# Autodesk Inventor assembly: finger-assembly
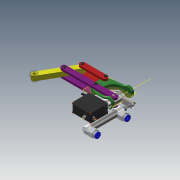
[picture p0: Inventor's stored thumbnail of the model, 180x180]
Saved by Autodesk Inventor 2017 (Build 210142000, 142)
## iProperties
Created: 2018-05-30
Part Number: finger-assembly
Document SubType Name: Assembly
Designer: Luiz Gustavo
Author: Luiz Gustavo
## Documents named in this file (14)
- C:\Users\Luiz Gustavo\Documents\Inventor\piano-robot\finger-assembly.iam
- C:\Users\Luiz Gustavo\Documents\Inventor\piano-robot\fingers-reference.ipt
- C:\Users\Luiz Gustavo\Documents\Inventor\piano-robot\biela-dedo-1.ipt
- C:\Users\Luiz Gustavo\Documents\Inventor\piano-robot\biela-dedo-2.ipt
- C:\Users\Luiz Gustavo\Documents\Inventor\piano-robot\biela-dedo-3.ipt
- C:\Users\Luiz Gustavo\Documents\Inventor\piano-robot\bloco-dedo-1.ipt
- C:\Users\Luiz Gustavo\Documents\Inventor\piano-robot\slider-1.ipt
- C:\Users\Luiz Gustavo\Documents\Inventor\piano-robot\tgy-901d.ipt
- C:\Users\Luiz Gustavo\Documents\Inventor\piano-robot\garfo-1.ipt
- C:\Users\Luiz Gustavo\Documents\Inventor\piano-robot\cylinderAssembly.iam
- C:\Users\Luiz Gustavo\Documents\Inventor\piano-robot\tip-protector.ipt
- C:\Users\Luiz Gustavo\Documents\Inventor\piano-robot\grabcad\AIRTAC 4V21008\PC602.ipt
- C:\Users\Luiz Gustavo\Documents\Inventor\piano-robot\finger-assembly\Design Accelerator\Bolted Connection1.iam
- C:\Users\Luiz Gustavo\Documents\Inventor\piano-robot\servo-metal-arm.ipt
## Components (14 placed, 13 different names)
1. fingers-reference:1 — Mate:1
2. biela-dedo-1:1 — Flush:1, Rotational:4, Rotational:5, Rigid:7
3. biela-dedo-2:1 — Flush:2, Rotational:3, Rotational:4, Mate:12, Mate:13
4. biela-dedo-3:1 — Flush:3, Rotational:2, Rotational:5, Transitional:1
5. bloco-dedo-1:1 — Flush:4, Rotational:2, Rotational:3, Mate:3, Mate:9, Mate:10
6. slider-1:1 — Mate:2, Flush:5, Mate:3, Rotational:6, Transitional:1
7. tgy-901d:1 — Mate:4, Angle:1, Flush:6, Mate:5
8. garfo-1:1 — Rigid:6, Rotational:6
9. cylinderAssembly:1 [sub-assembly] — Mate:5, Flush:7, Rigid:6, Rigid:8, Rigid:9
10. tip-protector:1 — Rigid:7
11. PC602:1 — Rigid:8
12. PC602:2 — Rigid:9
13. Bolted Connection:1 [sub-assembly] — Mate:12, Mate:13
14. servo-metal-arm:1 — Mate:9, Mate:10, Mate:11
## Relationships (28: Mate 10, Flush 7, RevoluteJoint 5, WeldJoint 4, Angle 1, Transitional 1)
- Flush:1: biela-dedo-1:1
- Flush:2: biela-dedo-2:1
- Flush:3: biela-dedo-3:1
- Flush:4: bloco-dedo-1:1
- Rotational:2 [RevoluteJoint]: biela-dedo-3:1 ↔ bloco-dedo-1:1
- Rotational:3 [RevoluteJoint]: biela-dedo-2:1 ↔ bloco-dedo-1:1
- Rotational:4 [RevoluteJoint]: biela-dedo-1:1 ↔ biela-dedo-2:1
- Rotational:5 [RevoluteJoint]: biela-dedo-1:1 ↔ biela-dedo-3:1
- Mate:1: fingers-reference:1
- Mate:2: slider-1:1
- Flush:5: slider-1:1
- Mate:3: bloco-dedo-1:1 ↔ slider-1:1
- Mate:4: tgy-901d:1
- Angle:1 (180 deg): tgy-901d:1
- Flush:6 (39.1 mm): tgy-901d:1
- Mate:5: tgy-901d:1 ↔ cylinderAssembly:1
- Flush:7 (48 mm): cylinderAssembly:1
- Rigid:6 [WeldJoint]: garfo-1:1 ↔ cylinderAssembly:1
- Rigid:7 [WeldJoint]: biela-dedo-1:1 ↔ tip-protector:1
- Rigid:8 [WeldJoint]: cylinderAssembly:1 ↔ PC602:1
- Rigid:9 [WeldJoint]: cylinderAssembly:1 ↔ PC602:2
- Mate:9: bloco-dedo-1:1 ↔ servo-metal-arm:1
- Mate:10: bloco-dedo-1:1 ↔ servo-metal-arm:1
- Mate:11: servo-metal-arm:1
- Mate:12: biela-dedo-2:1 ↔ Bolted Connection:1
- Mate:13: biela-dedo-2:1 ↔ Bolted Connection:1
- Rotational:6 [RevoluteJoint]: slider-1:1 ↔ garfo-1:1
- Transitional:1: biela-dedo-3:1 ↔ slider-1:1
